# Autodesk Inventor assembly: HexaBot
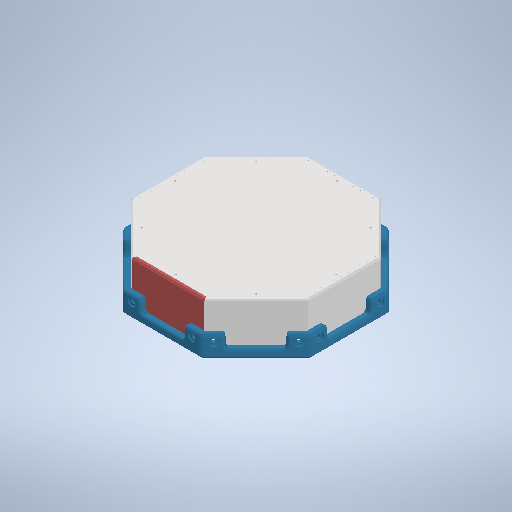
[picture p0: Inventor's stored thumbnail of the model, 512x512]
Saved by Autodesk Inventor 2025.1 (Build 291241020, 241B)
## iProperties
Created: 2024-08-28
Part Number: HexaBot
Document SubType Name: Assembly
Designer: SEON06
Author: SEON06
## Documents named in this file (4)
- C:\Users\daare\Documents\Inventor\HexaBot_s\HexaBot.iam
- C:\Users\daare\Documents\Inventor\HexaBot_s\Base.ipt
- C:\Users\daare\Documents\Inventor\HexaBot_s\Wall.ipt
- C:\Users\daare\Documents\Inventor\HexaBot_s\Cap.ipt
## Components (10 placed, 3 different names)
1. Base:1 — 메이트:1, 각도:1, 메이트:2, 메이트:3, 메이트:5, 메이트:6, 메이트:7, 메이트:8, 메이트:9, 메이트:10, 메이트:11, 메이트:12, 메이트:13, 메이트:14, 메이트:15, 메이트:16, 메이트:17, 메이트:18, 메이트:19, 메이트:20, 메이트:21
2. Wall:1 — 메이트:2, 메이트:3, 메이트:7, 대칭:2, 메이트:22
3. Wall:2 — 메이트:5, 메이트:6, 메이트:8, 대칭:1
4. Wall:3 — 메이트:9, 메이트:10, 메이트:11, 대칭:4
5. Wall:4 — 메이트:12, 메이트:17, 대칭:3
6. Wall:5 — 메이트:13, 메이트:18, 대칭:2
7. Wall:6 — 메이트:15, 메이트:20, 대칭:4
8. Wall:7 — 메이트:16, 메이트:19, 대칭:1
9. Wall:8 — 메이트:14, 메이트:21, 대칭:3, 메이트:23, 각도:2
10. Cap:1 — 메이트:22, 메이트:23, 각도:2
## Relationships (28: Mate 22, Symmetry 4, Angle 2)
- 메이트:1 [Mate]: Base:1
- 각도:1 [Angle] (0 deg): Base:1
- 메이트:2 [Mate]: Base:1 ↔ Wall:1
- 메이트:3 [Mate]: Base:1 ↔ Wall:1
- 메이트:5 [Mate]: Base:1 ↔ Wall:2
- 메이트:6 [Mate]: Base:1 ↔ Wall:2
- 메이트:7 [Mate]: Base:1 ↔ Wall:1
- 메이트:8 [Mate]: Base:1 ↔ Wall:2
- 메이트:9 [Mate]: Base:1 ↔ Wall:3
- 메이트:10 [Mate]: Base:1 ↔ Wall:3
- 메이트:11 [Mate]: Base:1 ↔ Wall:3
- 메이트:12 [Mate]: Base:1 ↔ Wall:4
- 메이트:13 [Mate]: Base:1 ↔ Wall:5
- 메이트:14 [Mate]: Base:1 ↔ Wall:8
- 메이트:15 [Mate]: Base:1 ↔ Wall:6
- 메이트:16 [Mate]: Base:1 ↔ Wall:7
- 메이트:17 [Mate]: Base:1 ↔ Wall:4
- 메이트:18 [Mate]: Base:1 ↔ Wall:5
- 메이트:19 [Mate]: Base:1 ↔ Wall:7
- 메이트:20 [Mate]: Base:1 ↔ Wall:6
- 메이트:21 [Mate]: Base:1 ↔ Wall:8
- 대칭:1 [Symmetry]: Wall:2 ↔ Wall:7
- 대칭:2 [Symmetry]: Wall:1 ↔ Wall:5
- 대칭:3 [Symmetry]: Wall:4 ↔ Wall:8
- 대칭:4 [Symmetry]: Wall:3 ↔ Wall:6
- 메이트:22 [Mate]: Wall:1 ↔ Cap:1
- 메이트:23 [Mate]: Wall:8 ↔ Cap:1
- 각도:2 [Angle] (0 deg): Wall:8 ↔ Cap:1
